# Autodesk Inventor assembly: penumatic and hyd
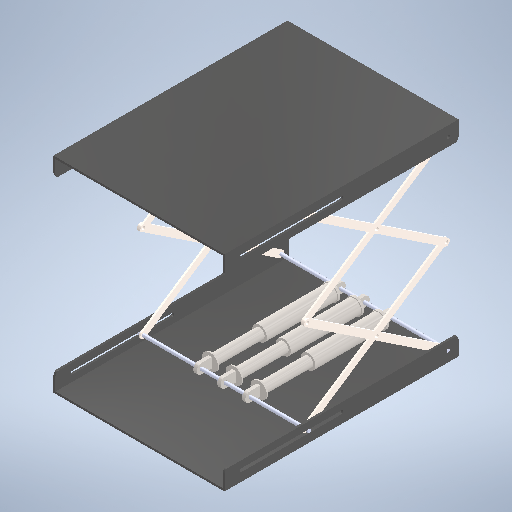
[picture p0: Inventor's stored thumbnail of the model, 512x512]
Saved by Autodesk Inventor 2025 (Build 290162000, 162)
## iProperties
Created: 2021-01-17
Part Number: penumatic and hyd
Document SubType Name: Assembly
Designer: mohamed salah
Author: mohamed salah
Sending System: SolidWorks 2016
Last Author: 91956
Last Saved: 2021-01-17
## Documents named in this file (10)
- C:\Users\mohamed salah\Desktop\4th year 2nd semester\hidrolik\project\penumatic and hyd.iam
- C:\Users\mohamed salah\Desktop\4th year 2nd semester\hidrolik\project\pneumatic-hydraulic-scissor-lift-mechanism-in-solidworks-1.snapshot.2\penumatic and hydraulic lift mechanism in solidworks\bar.ipt
- C:\Users\mohamed salah\Desktop\4th year 2nd semester\hidrolik\project\pneumatic-hydraulic-scissor-lift-mechanism-in-solidworks-1.snapshot.2\penumatic and hydraulic lift mechanism in solidworks\base 1.ipt
- C:\Users\mohamed salah\Desktop\4th year 2nd semester\hidrolik\project\pneumatic-hydraulic-scissor-lift-mechanism-in-solidworks-1.snapshot.2\penumatic and hydraulic lift mechanism in solidworks\Part3^Assem1.ipt
- C:\Users\mohamed salah\Desktop\4th year 2nd semester\hidrolik\project\pneumatic-hydraulic-scissor-lift-mechanism-in-solidworks-1.snapshot.2\penumatic and hydraulic lift mechanism in solidworks\Part4^Assem1.ipt
- C:\Users\mohamed salah\Desktop\4th year 2nd semester\hidrolik\project\pneumatic-hydraulic-scissor-lift-mechanism-in-solidworks-1.snapshot.2\penumatic and hydraulic lift mechanism in solidworks\Part5^Assem1.ipt
- C:\Users\mohamed salah\Desktop\4th year 2nd semester\hidrolik\project\pneumatic-hydraulic-scissor-lift-mechanism-in-solidworks-1.snapshot.2\penumatic and hydraulic lift mechanism in solidworks\Part5^Assem1_CPY1.ipt
- C:\Users\mohamed salah\Desktop\4th year 2nd semester\hidrolik\project\pneumatic-hydraulic-scissor-lift-mechanism-in-solidworks-1.snapshot.2\penumatic and hydraulic lift mechanism in solidworks\Part4^Assem1_CPY2.ipt
- C:\Users\mohamed salah\Desktop\4th year 2nd semester\hidrolik\project\pneumatic-hydraulic-scissor-lift-mechanism-in-solidworks-1.snapshot.2\penumatic and hydraulic lift mechanism in solidworks\Part5^Assem1_CPY2.ipt
- C:\Users\mohamed salah\Desktop\4th year 2nd semester\hidrolik\project\pneumatic-hydraulic-scissor-lift-mechanism-in-solidworks-1.snapshot.2\penumatic and hydraulic lift mechanism in solidworks\Part4^Assem1_CPY3.ipt
## Components (18 placed, 9 different names)
1. bar:1
2. base 1:1
3. bar:2
4. bar:3
5. bar:4
6. base 1:2
7. Part3^penumatic and hydraulic lift mechanism in solidworks:1 — Mate:2, Mate:5
8. Part3^penumatic and hydraulic lift mechanism in solidworks:2 — Mate:3, Mate:6
9. Part4^penumatic and hydraulic lift mechanism in solidworks:1
10. Part5^penumatic and hydraulic lift mechanism in solidworks:1
11. bar:5
12. bar:6
13. bar:7
14. bar:8
15. Part5^Assem1_CPY1:1 — Mate:2, Mate:4
16. Part4^Assem1_CPY2:1 — Mate:3, Mate:4
17. Part5^Assem1_CPY2:1 — Mate:5, Mate:7
18. Part4^Assem1_CPY3:1 — Mate:6, Mate:7
## Relationships (6: Mate 6)
- Mate:2: Part3^penumatic and hydraulic lift mechanism in solidworks:1 ↔ Part5^Assem1_CPY1:1
- Mate:3: Part3^penumatic and hydraulic lift mechanism in solidworks:2 ↔ Part4^Assem1_CPY2:1
- Mate:4: Part5^Assem1_CPY1:1 ↔ Part4^Assem1_CPY2:1
- Mate:5: Part3^penumatic and hydraulic lift mechanism in solidworks:1 ↔ Part5^Assem1_CPY2:1
- Mate:6: Part3^penumatic and hydraulic lift mechanism in solidworks:2 ↔ Part4^Assem1_CPY3:1
- Mate:7: Part5^Assem1_CPY2:1 ↔ Part4^Assem1_CPY3:1
